# Autodesk Inventor assembly: drive_right
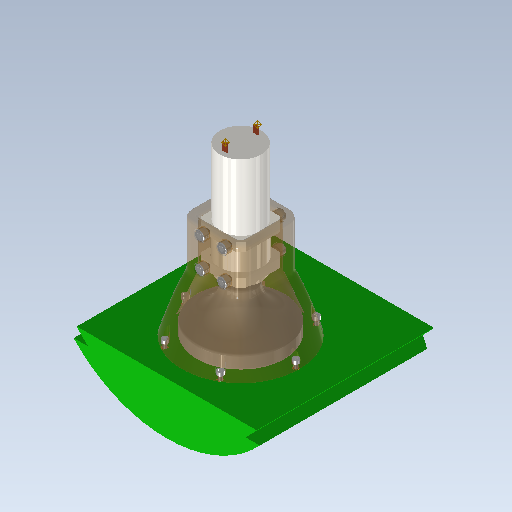
[picture p0: Inventor's stored thumbnail of the model, 512x512]
Saved by Autodesk Inventor 2020.2 (Build 242310000, 310)
## iProperties
Created: 2019-10-27
Part Number: drive_right
Document SubType Name: Assembly
Designer: agmle
Mass: 1094.26 g
Surface Area: 2147.54 cm^2
Volume: 971.44 cm^3
Density: 1.12644 g/cm^3
Author: agmle
## Documents named in this file (15)
- D:\syncthing\rwsir-rc7py\projects\CreekFleet\CreekFleet_AutoBuoy\Mechanical CAD\propulsion\drive_right.iam
- D:\syncthing\rwsir-rc7py\projects\CreekFleet\CreekFleet_AutoBuoy\Mechanical CAD\propulsion\impeller_right.ipt
- D:\syncthing\rwsir-rc7py\projects\CreekFleet\CreekFleet_AutoBuoy\Mechanical CAD\propulsion\bearing\6138k63.iam
- D:\syncthing\rwsir-rc7py\projects\CreekFleet\CreekFleet_AutoBuoy\Mechanical CAD\propulsion\shaft.ipt
- D:\syncthing\rwsir-rc7py\projects\CreekFleet\CreekFleet_AutoBuoy\Mechanical CAD\propulsion\6x10mm magnet.ipt
- D:\syncthing\rwsir-rc7py\projects\CreekFleet\CreekFleet_AutoBuoy\Mechanical CAD\propulsion\drive_disc.ipt
- \\rackstation\media\documents\Inventor\Content Center Files\R2020\en-US\ANSI B18.3.6M(01)\ANSI B18.3.6M - M3x0.5 x 5(2).ipt
- D:\syncthing\rwsir-rc7py\projects\CreekFleet\CreekFleet_AutoBuoy\Mechanical CAD\propulsion\rs550_p60s-4-57.ipt
- D:\syncthing\rwsir-rc7py\projects\CreekFleet\CreekFleet_AutoBuoy\Mechanical CAD\propulsion\motor_mount.ipt
- \\rackstation\media\documents\Inventor\Content Center Files\R2020\en-US\ANSI B18.3(05)\ANSI B18.3 - 10-32 UNF - 0.5(31).ipt
- D:\syncthing\rwsir-rc7py\projects\CreekFleet\CreekFleet_AutoBuoy\Mechanical CAD\propulsion\inner_drive_right.ipt
- D:\syncthing\rwsir-rc7py\projects\CreekFleet\CreekFleet_AutoBuoy\Mechanical CAD\hardware\94459A140_BRASS HEAT-SET INSERT FOR PLASTIC.ipt
- D:\syncthing\rwsir-rc7py\projects\CreekFleet\CreekFleet_AutoBuoy\Mechanical CAD\propulsion\intake_cover.ipt
- \\rackstation\media\documents\Inventor\Content Center Files\R2020\en-US\ANSI B18.3.1M(6)\ANSI B18.3.1M - M3x0.5 x 8(1).ipt
- D:\syncthing\rwsir-rc7py\projects\CreekFleet\CreekFleet_AutoBuoy\Mechanical CAD\propulsion\discharge_sealant.ipt
## Components (54 placed, 14 different names)
1. 6138k63:1 [sub-assembly] — Insert:82
2. 6138k63:2 [sub-assembly] — Insert:80, Insert:81, Mate:11
3. shaft:1 — Insert:81, Insert:82, Cylindrical:1
4. impeller_right:1 — Insert:13, Insert:14, Insert:15, Insert:16, Insert:17, Insert:18, Cylindrical:1, Mate:11, Mate:12
5. 6x10mm magnet:1 — Insert:17
6. 6x10mm magnet:2 — Insert:18
7. 6x10mm magnet:3 — Insert:13
8. 6x10mm magnet:4 — Insert:14
9. 6x10mm magnet:5 — Insert:15
10. 6x10mm magnet:6 — Insert:16
11. Broached Hexagon Socket Set Screw - Flat Point - Metric M3x0.5 x 5:1 — Insert:20
12. Broached Hexagon Socket Set Screw - Flat Point - Metric M3x0.5 x 5:2 — Insert:21
13. drive_disc:1 — Insert:7, Insert:8, Insert:9, Insert:10, Insert:11, Insert:12, Insert:20, Insert:21, Mate:4, Mate:6, Flush:1, Mate:12
14. 6x10mm magnet:7 — Insert:7
15. 6x10mm magnet:8 — Insert:11
16. 6x10mm magnet:9 — Insert:12
17. 6x10mm magnet:10 — Insert:8
18. 6x10mm magnet:11 — Insert:9
19. 6x10mm magnet:12 — Insert:10
20. Forged Socket Head Cap Screw - Metric M3x0.5 x 8:2 — Insert:102
21. Forged Socket Head Cap Screw - Metric M3x0.5 x 8:3 — Insert:103
22. Forged Socket Head Cap Screw - Metric M3x0.5 x 8:4 — Insert:104
23. Forged Socket Head Cap Screw - Metric M3x0.5 x 8:5 — Insert:105
24. Forged Socket Head Cap Screw - Metric M3x0.5 x 8:6 — Insert:106
25. Forged Socket Head Cap Screw - Metric M3x0.5 x 8:7 — Insert:101
26. 94459A140_BRASS HEAT-SET INSERT FOR PLASTIC:6 — Insert:93, Mate:17
27. 94459A140_BRASS HEAT-SET INSERT FOR PLASTIC:7 — Insert:92
28. 94459A140_BRASS HEAT-SET INSERT FOR PLASTIC:8 — Insert:94
29. 94459A140_BRASS HEAT-SET INSERT FOR PLASTIC:9 — Insert:95
30. 94459A140_BRASS HEAT-SET INSERT FOR PLASTIC:10 — Insert:91
31. 94459A140_BRASS HEAT-SET INSERT FOR PLASTIC:11 — Insert:90
32. rs550_p60s-4-57:1 — Mate:4, Mate:6, Flush:1, Mate:13, Mate:14, Mate:15
33. motor_mount:1 — Insert:72, Insert:73, Insert:74, Insert:75, Insert:76, Insert:77, Insert:78, Insert:79, Mate:15, Mate:16, Mate:17, Insert:101, Insert:102, Insert:103, Insert:104, Insert:105, Insert:106
34. Hexagon Socket Head Cap Screw - Inch 10-32 UNF - 0.5:1 — Insert:77
35. Hexagon Socket Head Cap Screw - Inch 10-32 UNF - 0.5:2 — Insert:76
36. Hexagon Socket Head Cap Screw - Inch 10-32 UNF - 0.5:3 — Insert:78
37. Hexagon Socket Head Cap Screw - Inch 10-32 UNF - 0.5:4 — Insert:79
38. Hexagon Socket Head Cap Screw - Inch 10-32 UNF - 0.5:5 — Insert:72, Mate:14
39. Hexagon Socket Head Cap Screw - Inch 10-32 UNF - 0.5:6 — Insert:73
40. Hexagon Socket Head Cap Screw - Inch 10-32 UNF - 0.5:7 — Insert:75
41. Hexagon Socket Head Cap Screw - Inch 10-32 UNF - 0.5:8 — Insert:74, Mate:13
42. discharge_sealant:1 — Mate:18, Mate:19
43. Forged Socket Head Cap Screw - Metric M3x0.5 x 8:1 — Insert:96
44. Forged Socket Head Cap Screw - Metric M3x0.5 x 8:8 — Insert:100
45. Forged Socket Head Cap Screw - Metric M3x0.5 x 8:9 — Insert:99
46. Forged Socket Head Cap Screw - Metric M3x0.5 x 8:10 — Insert:98
47. Forged Socket Head Cap Screw - Metric M3x0.5 x 8:11 — Insert:97
48. inner_drive_right:1 — Mate:8, Mate:9, Mate:10, Insert:80, Mate:16, Insert:83, Insert:84, Insert:85, Insert:86, Insert:87, Insert:88, Insert:89, Insert:90, Insert:91, Insert:92, Insert:93, Insert:94, Insert:95, Mate:18, Mate:19
49. 94459A140_BRASS HEAT-SET INSERT FOR PLASTIC:1 — Insert:87
50. 94459A140_BRASS HEAT-SET INSERT FOR PLASTIC:2 — Insert:86
51. 94459A140_BRASS HEAT-SET INSERT FOR PLASTIC:3 — Insert:84
52. 94459A140_BRASS HEAT-SET INSERT FOR PLASTIC:4 — Insert:85
53. 94459A140_BRASS HEAT-SET INSERT FOR PLASTIC:5 — Insert:83
54. intake_cover:1 — Insert:88, Insert:89, Insert:96, Insert:97, Insert:98, Insert:99, Insert:100
## Relationships (65: Insert 49, Mate 14, CylindricalJoint 1, Flush 1)
- Insert:7: drive_disc:1 ↔ 6x10mm magnet:7
- Insert:8: drive_disc:1 ↔ 6x10mm magnet:10
- Insert:9: drive_disc:1 ↔ 6x10mm magnet:11
- Insert:10: drive_disc:1 ↔ 6x10mm magnet:12
- Insert:11: drive_disc:1 ↔ 6x10mm magnet:8
- Insert:12: drive_disc:1 ↔ 6x10mm magnet:9
- Insert:13: impeller_right:1 ↔ 6x10mm magnet:3
- Insert:14: impeller_right:1 ↔ 6x10mm magnet:4
- Insert:15: impeller_right:1 ↔ 6x10mm magnet:5
- Insert:16: impeller_right:1 ↔ 6x10mm magnet:6
- Insert:17: impeller_right:1 ↔ 6x10mm magnet:1
- Insert:18: impeller_right:1 ↔ 6x10mm magnet:2
- Insert:20: Broached Hexagon Socket Set Screw - Flat Point - Metric M3x0.5 x 5:1 ↔ drive_disc:1
- Insert:21: Broached Hexagon Socket Set Screw - Flat Point - Metric M3x0.5 x 5:2 ↔ drive_disc:1
- Mate:4: drive_disc:1 ↔ rs550_p60s-4-57:1
- Mate:6: drive_disc:1 ↔ rs550_p60s-4-57:1
- Insert:72: motor_mount:1 ↔ Hexagon Socket Head Cap Screw - Inch 10-32 UNF - 0.5:5
- Insert:73: motor_mount:1 ↔ Hexagon Socket Head Cap Screw - Inch 10-32 UNF - 0.5:6
- Insert:74: motor_mount:1 ↔ Hexagon Socket Head Cap Screw - Inch 10-32 UNF - 0.5:8
- Insert:75: motor_mount:1 ↔ Hexagon Socket Head Cap Screw - Inch 10-32 UNF - 0.5:7
- Insert:76: motor_mount:1 ↔ Hexagon Socket Head Cap Screw - Inch 10-32 UNF - 0.5:2
- Insert:77: motor_mount:1 ↔ Hexagon Socket Head Cap Screw - Inch 10-32 UNF - 0.5:1
- Insert:78: motor_mount:1 ↔ Hexagon Socket Head Cap Screw - Inch 10-32 UNF - 0.5:3
- Insert:79: motor_mount:1 ↔ Hexagon Socket Head Cap Screw - Inch 10-32 UNF - 0.5:4
- Mate:8: inner_drive_right:1
- Mate:9: inner_drive_right:1
- Mate:10: inner_drive_right:1
- Insert:80: 6138k63:2 ↔ inner_drive_right:1
- Insert:81: 6138k63:2 ↔ shaft:1
- Insert:82: 6138k63:1 ↔ shaft:1
- Cylindrical:1: shaft:1 ↔ impeller_right:1
- Mate:11: 6138k63:2 ↔ impeller_right:1
- Flush:1: drive_disc:1 ↔ rs550_p60s-4-57:1
- Mate:12: impeller_right:1 ↔ drive_disc:1
- Mate:13: rs550_p60s-4-57:1 ↔ Hexagon Socket Head Cap Screw - Inch 10-32 UNF - 0.5:8
- Mate:14: rs550_p60s-4-57:1 ↔ Hexagon Socket Head Cap Screw - Inch 10-32 UNF - 0.5:5
- Mate:15: rs550_p60s-4-57:1 ↔ motor_mount:1
- Mate:16: motor_mount:1 ↔ inner_drive_right:1
- Insert:83: inner_drive_right:1 ↔ 94459A140_BRASS HEAT-SET INSERT FOR PLASTIC:5
- Insert:84: inner_drive_right:1 ↔ 94459A140_BRASS HEAT-SET INSERT FOR PLASTIC:3
- Insert:85: inner_drive_right:1 ↔ 94459A140_BRASS HEAT-SET INSERT FOR PLASTIC:4
- Insert:86: inner_drive_right:1 ↔ 94459A140_BRASS HEAT-SET INSERT FOR PLASTIC:2
- Insert:87: inner_drive_right:1 ↔ 94459A140_BRASS HEAT-SET INSERT FOR PLASTIC:1
- Insert:88: inner_drive_right:1 ↔ intake_cover:1
- Insert:89: inner_drive_right:1 ↔ intake_cover:1
- Insert:90: 94459A140_BRASS HEAT-SET INSERT FOR PLASTIC:11 ↔ inner_drive_right:1
- Insert:91: 94459A140_BRASS HEAT-SET INSERT FOR PLASTIC:10 ↔ inner_drive_right:1
- Insert:92: 94459A140_BRASS HEAT-SET INSERT FOR PLASTIC:7 ↔ inner_drive_right:1
- Insert:93: 94459A140_BRASS HEAT-SET INSERT FOR PLASTIC:6 ↔ inner_drive_right:1
- Insert:94: 94459A140_BRASS HEAT-SET INSERT FOR PLASTIC:8 ↔ inner_drive_right:1
- Insert:95: 94459A140_BRASS HEAT-SET INSERT FOR PLASTIC:9 ↔ inner_drive_right:1
- Mate:17: 94459A140_BRASS HEAT-SET INSERT FOR PLASTIC:6 ↔ motor_mount:1
- Insert:96: Forged Socket Head Cap Screw - Metric M3x0.5 x 8:1 ↔ intake_cover:1
- Insert:97: Forged Socket Head Cap Screw - Metric M3x0.5 x 8:11 ↔ intake_cover:1
- Insert:98: Forged Socket Head Cap Screw - Metric M3x0.5 x 8:10 ↔ intake_cover:1
- Insert:99: Forged Socket Head Cap Screw - Metric M3x0.5 x 8:9 ↔ intake_cover:1
- Insert:100: Forged Socket Head Cap Screw - Metric M3x0.5 x 8:8 ↔ intake_cover:1
- Insert:101: Forged Socket Head Cap Screw - Metric M3x0.5 x 8:7 ↔ motor_mount:1
- Insert:102: Forged Socket Head Cap Screw - Metric M3x0.5 x 8:2 ↔ motor_mount:1
- Insert:103: Forged Socket Head Cap Screw - Metric M3x0.5 x 8:3 ↔ motor_mount:1
- Insert:104: Forged Socket Head Cap Screw - Metric M3x0.5 x 8:4 ↔ motor_mount:1
- Insert:105: Forged Socket Head Cap Screw - Metric M3x0.5 x 8:5 ↔ motor_mount:1
- Insert:106: Forged Socket Head Cap Screw - Metric M3x0.5 x 8:6 ↔ motor_mount:1
- Mate:18: discharge_sealant:1 ↔ inner_drive_right:1
- Mate:19: discharge_sealant:1 ↔ inner_drive_right:1
